# Autodesk Inventor assembly: A004
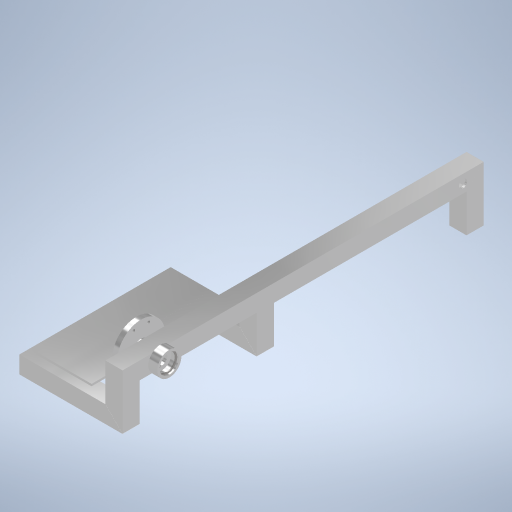
[picture p0: Inventor's stored thumbnail of the model, 512x512]
Saved by Autodesk Inventor 2023 (Build 270158000, 158)
## iProperties
Created: 2022-08-29
Part Number: A004
Document SubType Name: Assembly
Designer: D.C. Eksteen
Author: D.C. Eksteen
Title: LEFT REAR FRAME ASSEMBLY
## Documents named in this file (13)
- C:\Users\dylan\Desktop\Skripsie-2022\Design\CAD\LEFT FRAME.iam
- C:\Users\dylan\Desktop\Skripsie-2022\Design\CAD\LEFT TOP TUBE.ipt
- C:\Users\dylan\Desktop\Skripsie-2022\Design\CAD\RISER.ipt
- C:\Users\dylan\Desktop\Skripsie-2022\Design\CAD\REAR RISER BRAKE.ipt
- C:\Users\dylan\Desktop\Skripsie-2022\Design\CAD\CONTROL RISER.ipt
- C:\Users\dylan\Desktop\Skripsie-2022\Design\CAD\BRAKE BRACKET.ipt
- C:\Users\dylan\Desktop\Skripsie-2022\Design\CAD\CONTROL RISER FRONT.ipt
- C:\Users\dylan\Desktop\Skripsie-2022\Design\CAD\BRAKE MOUNT PLATE.ipt
- C:\Users\dylan\Desktop\Skripsie-2022\Design\CAD\BRAKE MOUNT PLATE 2.ipt
- C:\Users\dylan\Desktop\Skripsie\WORKSHOP\PARTS 2\REAR FRAME\BRAKE RISER 2.ipt
- C:\Users\dylan\Desktop\Skripsie-2022\Design\CAD\472-028.ipt
- C:\Users\dylan\Desktop\Skripsie-2022\Design\CAD\BEARING AND MAGNET DISC MOUNT.ipt
- C:\Users\dylan\Desktop\Skripsie-2022\Design\CAD\BEARING AND MAGNET DISC MOUNT BRACKET.ipt
## Components (12 placed, 12 different names)
1. LEFT TOP TUBE:1 — Mate:5, Flush:2, Mate:6, Mate:11, Flush:3, Mate:12, Mate:25, Mate:27, Mate:28, Mate:29, Angle:2
2. RISER:2 — Mate:5, Flush:2, Mate:6
3. UNI 7437 28:1
4. REAR RISER BRAKE:1 — Mate:11, Flush:3, Mate:12, Mate:23, Flush:10, Mate:24
5. CONTROL RISER:1 — Mate:23, Flush:10, Mate:24
6. BRAKE BRACKET:1
7. CONTROL RISER FRONT:1
8. BRAKE MOUNT PLATE:1
9. BRAKE MOUNT PLATE 2:1
10. BRAKE RISER 2:1 — Mate:25
11. BEARING AND MAGNET DISC MOUNT:1 — Tangent:1, Tangent:2, Mate:26, Angle:2
12. BEARING AND MAGNET DISC MOUNT BRACKET:1 — Tangent:1, Tangent:2, Mate:26, Mate:27, Mate:28, Mate:29
## Relationships (32: Mate 19, Flush 9, Angle 2, Tangent 2)
- Mate:5: LEFT TOP TUBE:1 ↔ RISER:2
- Flush:2: LEFT TOP TUBE:1 ↔ RISER:2
- Mate:6: LEFT TOP TUBE:1 ↔ RISER:2
- Mate:11: LEFT TOP TUBE:1 ↔ REAR RISER BRAKE:1
- Flush:3: LEFT TOP TUBE:1 ↔ REAR RISER BRAKE:1
- Mate:12: LEFT TOP TUBE:1 ↔ REAR RISER BRAKE:1
- [Mate]: CONTROL RISER:1 ↔ BRAKE BRACKET:1
- [Flush]: CONTROL RISER:1 ↔ BRAKE BRACKET:1
- [Mate]: CONTROL RISER:1 ↔ BRAKE BRACKET:1
- [Mate]: BRAKE BRACKET:1 ↔ CONTROL RISER FRONT:1
- [Flush]: BRAKE BRACKET:1 ↔ CONTROL RISER FRONT:1
- [Mate]: BRAKE BRACKET:1 ↔ CONTROL RISER FRONT:1
- [Mate]: CONTROL RISER:1 ↔ BRAKE MOUNT PLATE:1
- [Angle] (0 deg): BRAKE BRACKET:1 ↔ BRAKE MOUNT PLATE:1
- [Flush] (12.5 mm): BRAKE BRACKET:1 ↔ BRAKE MOUNT PLATE:1
- [Flush] (12.5 mm): CONTROL RISER:1 ↔ BRAKE MOUNT PLATE:1
- [Mate]: CONTROL RISER FRONT:1 ↔ BRAKE MOUNT PLATE 2:1
- [Flush]: BRAKE MOUNT PLATE:1 ↔ BRAKE MOUNT PLATE 2:1
- [Mate]: BRAKE MOUNT PLATE:1 ↔ BRAKE MOUNT PLATE 2:1
- [Mate]: CONTROL RISER FRONT:1 ↔ BRAKE RISER 2:1
- [Flush]: CONTROL RISER FRONT:1 ↔ BRAKE RISER 2:1
- Mate:23: REAR RISER BRAKE:1 ↔ CONTROL RISER:1
- Flush:10: REAR RISER BRAKE:1 ↔ CONTROL RISER:1
- Mate:24: REAR RISER BRAKE:1 ↔ CONTROL RISER:1
- Mate:25: LEFT TOP TUBE:1 ↔ BRAKE RISER 2:1
- Tangent:1: BEARING AND MAGNET DISC MOUNT:1 ↔ BEARING AND MAGNET DISC MOUNT BRACKET:1
- Tangent:2: BEARING AND MAGNET DISC MOUNT:1 ↔ BEARING AND MAGNET DISC MOUNT BRACKET:1
- Mate:26: BEARING AND MAGNET DISC MOUNT:1 ↔ BEARING AND MAGNET DISC MOUNT BRACKET:1
- Mate:27: LEFT TOP TUBE:1 ↔ BEARING AND MAGNET DISC MOUNT BRACKET:1
- Mate:28: LEFT TOP TUBE:1 ↔ BEARING AND MAGNET DISC MOUNT BRACKET:1
- Mate:29: LEFT TOP TUBE:1 ↔ BEARING AND MAGNET DISC MOUNT BRACKET:1
- Angle:2 (90 deg): LEFT TOP TUBE:1 ↔ BEARING AND MAGNET DISC MOUNT:1
